# Autodesk Inventor assembly: Rack-RAM
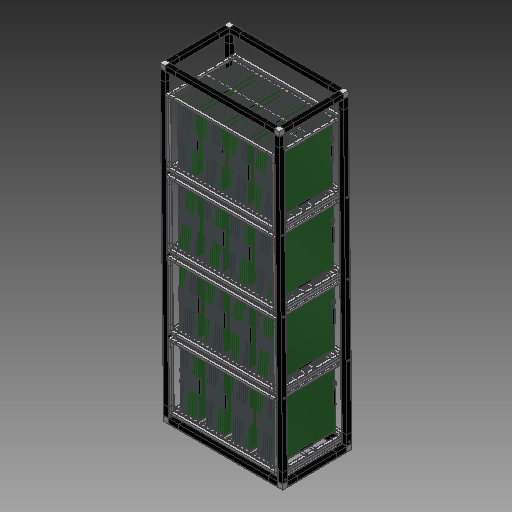
[picture p0: Inventor's stored thumbnail of the model, 512x512]
Saved by Autodesk Inventor 2018 (Build 220112000, 112)
## iProperties
Created: 2025-02-17
Part Number: Rack-RAM
Material: Všeobecné
Document SubType Name: Assembly
Designer: Jozko Mrkvicka
Author: Jozko Mrkvicka
## Documents named in this file (10)
- D:\05_Projekty\Projects_Inventor\Haluska9000\Rack-RAM.iam
- D:\05_Projekty\Projects_Inventor\Haluska9000\Profile-Connector\Profile-Connector#30x30xCorner.ipt
- D:\05_Projekty\Projects_Inventor\Haluska9000\Profile-Connector.ipt
- D:\05_Projekty\Projects_Inventor\Haluska9000\Cabinet-FerriteCore.iam
- D:\05_Projekty\Projects_Inventor\Haluska9000\Profile-Square-Black\Profile-Square#Rack-Ram-Height.ipt
- D:\05_Projekty\Projects_Inventor\Haluska9000\Profile-Square-Black.ipt
- D:\05_Projekty\Projects_Inventor\Haluska9000\Profile-Square-Black\Profile-Square#Rack-Ram-Width.ipt
- D:\05_Projekty\Projects_Inventor\Haluska9000\Profile-Square-Black\Profile-Square#Rack-Ram-Length.ipt
- D:\05_Projekty\Projects_Inventor\Haluska9000\Profile-T\Profile-T#Rack-Ram.ipt
- D:\05_Projekty\Projects_Inventor\Haluska9000\Profile-T.ipt
## Components (32 placed, 6 different names)
1. Cabinet-FerriteCore:1 [sub-assembly] — Proti sobě:627, Proti sobě:628, Stejný směr:50, Stejný směr:51
2. Profile-Connector#30x30xCorner:11 — Proti sobě:560, Proti sobě:561, Proti sobě:562, Proti sobě:572, Proti sobě:573, Proti sobě:574, Proti sobě:590, Proti sobě:591, Proti sobě:592
3. Profile-Connector#30x30xCorner:12 — Proti sobě:569, Proti sobě:570, Proti sobě:571, Proti sobě:575, Proti sobě:576, Proti sobě:577
4. Profile-Connector#30x30xCorner:13 — Proti sobě:581, Proti sobě:582, Proti sobě:583, Proti sobě:587, Proti sobě:588, Proti sobě:589
5. Profile-Connector#30x30xCorner:14 — Proti sobě:578, Proti sobě:579, Proti sobě:580, Proti sobě:584, Proti sobě:585, Proti sobě:586, Proti sobě:646, Proti sobě:647, Proti sobě:648
6. Profile-Square#Rack-Ram-Height:1 — Proti sobě:560, Proti sobě:561, Proti sobě:562, Proti sobě:581, Proti sobě:582, Proti sobě:583, Proti sobě:624, Stejný směr:36, Proti sobě:625, Stejný směr:40, Proti sobě:639, Proti sobě:640, Stejný směr:45, Stejný směr:46
7. Profile-Square#Rack-Ram-Height:3 — Proti sobě:569, Proti sobě:570, Proti sobě:571, Proti sobě:578, Proti sobě:579, Proti sobě:580, Proti sobě:623, Stejný směr:35, Proti sobě:626, Stejný směr:39, Proti sobě:629, Proti sobě:630, Proti sobě:637, Proti sobě:638, Stejný směr:43, Stejný směr:44, Proti sobě:641, Proti sobě:642
8. Profile-Square#Rack-Ram-Length:5 — Proti sobě:572, Proti sobě:573, Proti sobě:574, Proti sobě:620, Proti sobě:621, Proti sobě:622
9. Profile-Square#Rack-Ram-Length:6 — Proti sobě:575, Proti sobě:576, Proti sobě:577
10. Profile-Square#Rack-Ram-Length:11
11. Profile-Square#Rack-Ram-Length:12 — Proti sobě:646, Proti sobě:647, Proti sobě:648
12. Profile-Square#Rack-Ram-Width:7 — Proti sobě:584, Proti sobě:585, Proti sobě:586, Proti sobě:587, Proti sobě:588, Proti sobě:589
13. Profile-Square#Rack-Ram-Width:8 — Proti sobě:590, Proti sobě:591, Proti sobě:592
14. Profile-Square#Rack-Ram-Width:13
15. Profile-Square#Rack-Ram-Width:14 — Proti sobě:643, Proti sobě:644, Proti sobě:645
16. Profile-Connector#30x30xCorner:15
17. Profile-Connector#30x30xCorner:16 — Proti sobě:643, Proti sobě:644, Proti sobě:645
18. Profile-Connector#30x30xCorner:17 — Proti sobě:620, Proti sobě:621, Proti sobě:622, Proti sobě:631, Proti sobě:632, Proti sobě:633
19. Profile-Connector#30x30xCorner:18 — Proti sobě:634, Proti sobě:635, Proti sobě:636
20. Profile-T#Rack-Ram:1 — Proti sobě:623, Stejný směr:35, Stejný směr:37, Proti sobě:627, Proti sobě:628, Proti sobě:629
21. Profile-T#Rack-Ram:2 — Proti sobě:624, Stejný směr:36, Stejný směr:37
22. Profile-T#Rack-Ram:3 — Proti sobě:626, Stejný směr:39, Proti sobě:630, Proti sobě:649
23. Profile-T#Rack-Ram:4 — Proti sobě:625, Stejný směr:40
24. Profile-Square#Rack-Ram-Height:15 — Proti sobě:631, Proti sobě:632, Proti sobě:633
25. Profile-Square#Rack-Ram-Height:16 — Proti sobě:634, Proti sobě:635, Proti sobě:636
26. Profile-T#Rack-Ram:5 — Proti sobě:638, Stejný směr:43, Proti sobě:641, Proti sobě:650
27. Profile-T#Rack-Ram:6 — Proti sobě:640, Stejný směr:46
28. Profile-T#Rack-Ram:7 — Proti sobě:637, Stejný směr:44, Proti sobě:642, Proti sobě:651
29. Profile-T#Rack-Ram:8 — Proti sobě:639, Stejný směr:45
30. Cabinet-FerriteCore:2 [sub-assembly] — Proti sobě:650, Stejný směr:48, Stejný směr:49, Stejný směr:52, Stejný směr:53
31. Cabinet-FerriteCore:3 [sub-assembly] — Proti sobě:649, Stejný směr:49, Stejný směr:50, Stejný směr:51, Stejný směr:52
32. Cabinet-FerriteCore:4 [sub-assembly] — Proti sobě:651, Stejný směr:48, Stejný směr:53
## Relationships (92: Mate 74, Flush 18)
- Proti sobě:560 [Mate]: Profile-Connector#30x30xCorner:11 ↔ Profile-Square#Rack-Ram-Height:1
- Proti sobě:561 [Mate]: Profile-Connector#30x30xCorner:11 ↔ Profile-Square#Rack-Ram-Height:1
- Proti sobě:562 [Mate]: Profile-Connector#30x30xCorner:11 ↔ Profile-Square#Rack-Ram-Height:1
- Proti sobě:569 [Mate]: Profile-Connector#30x30xCorner:12 ↔ Profile-Square#Rack-Ram-Height:3
- Proti sobě:570 [Mate]: Profile-Connector#30x30xCorner:12 ↔ Profile-Square#Rack-Ram-Height:3
- Proti sobě:571 [Mate]: Profile-Connector#30x30xCorner:12 ↔ Profile-Square#Rack-Ram-Height:3
- Proti sobě:572 [Mate]: Profile-Connector#30x30xCorner:11 ↔ Profile-Square#Rack-Ram-Length:5
- Proti sobě:573 [Mate]: Profile-Connector#30x30xCorner:11 ↔ Profile-Square#Rack-Ram-Length:5
- Proti sobě:574 [Mate]: Profile-Connector#30x30xCorner:11 ↔ Profile-Square#Rack-Ram-Length:5
- Proti sobě:575 [Mate]: Profile-Connector#30x30xCorner:12 ↔ Profile-Square#Rack-Ram-Length:6
- Proti sobě:576 [Mate]: Profile-Connector#30x30xCorner:12 ↔ Profile-Square#Rack-Ram-Length:6
- Proti sobě:577 [Mate]: Profile-Connector#30x30xCorner:12 ↔ Profile-Square#Rack-Ram-Length:6
- Proti sobě:578 [Mate]: Profile-Connector#30x30xCorner:14 ↔ Profile-Square#Rack-Ram-Height:3
- Proti sobě:579 [Mate]: Profile-Connector#30x30xCorner:14 ↔ Profile-Square#Rack-Ram-Height:3
- Proti sobě:580 [Mate]: Profile-Connector#30x30xCorner:14 ↔ Profile-Square#Rack-Ram-Height:3
- Proti sobě:581 [Mate]: Profile-Connector#30x30xCorner:13 ↔ Profile-Square#Rack-Ram-Height:1
- Proti sobě:582 [Mate]: Profile-Connector#30x30xCorner:13 ↔ Profile-Square#Rack-Ram-Height:1
- Proti sobě:583 [Mate]: Profile-Connector#30x30xCorner:13 ↔ Profile-Square#Rack-Ram-Height:1
- Proti sobě:584 [Mate]: Profile-Connector#30x30xCorner:14 ↔ Profile-Square#Rack-Ram-Width:7
- Proti sobě:585 [Mate]: Profile-Connector#30x30xCorner:14 ↔ Profile-Square#Rack-Ram-Width:7
- Proti sobě:586 [Mate]: Profile-Connector#30x30xCorner:14 ↔ Profile-Square#Rack-Ram-Width:7
- Proti sobě:587 [Mate]: Profile-Connector#30x30xCorner:13 ↔ Profile-Square#Rack-Ram-Width:7
- Proti sobě:588 [Mate]: Profile-Connector#30x30xCorner:13 ↔ Profile-Square#Rack-Ram-Width:7
- Proti sobě:589 [Mate]: Profile-Connector#30x30xCorner:13 ↔ Profile-Square#Rack-Ram-Width:7
- Proti sobě:590 [Mate]: Profile-Connector#30x30xCorner:11 ↔ Profile-Square#Rack-Ram-Width:8
- Proti sobě:591 [Mate]: Profile-Connector#30x30xCorner:11 ↔ Profile-Square#Rack-Ram-Width:8
- Proti sobě:592 [Mate]: Profile-Connector#30x30xCorner:11 ↔ Profile-Square#Rack-Ram-Width:8
- [Mate]: Profile-Square#Rack-Ram-Length:11 ↔ Profile-Connector#30x30xCorner:15
- [Mate]: Profile-Square#Rack-Ram-Length:11 ↔ Profile-Connector#30x30xCorner:15
- [Mate]: Profile-Square#Rack-Ram-Length:11 ↔ Profile-Connector#30x30xCorner:15
- [Mate]: Profile-Square#Rack-Ram-Length:12 ↔ Profile-Connector#30x30xCorner:16
- [Mate]: Profile-Square#Rack-Ram-Length:12 ↔ Profile-Connector#30x30xCorner:16
- [Mate]: Profile-Square#Rack-Ram-Length:12 ↔ Profile-Connector#30x30xCorner:16
- [Mate]: Profile-Square#Rack-Ram-Width:13 ↔ Profile-Connector#30x30xCorner:18
- [Mate]: Profile-Square#Rack-Ram-Width:13 ↔ Profile-Connector#30x30xCorner:18
- [Mate]: Profile-Square#Rack-Ram-Width:13 ↔ Profile-Connector#30x30xCorner:18
- [Mate]: Profile-Square#Rack-Ram-Width:13 ↔ Profile-Connector#30x30xCorner:17
- [Mate]: Profile-Square#Rack-Ram-Width:13 ↔ Profile-Connector#30x30xCorner:17
- [Mate]: Profile-Square#Rack-Ram-Width:13 ↔ Profile-Connector#30x30xCorner:17
- [Mate]: Profile-Square#Rack-Ram-Width:14 ↔ Profile-Connector#30x30xCorner:15
- [Mate]: Profile-Square#Rack-Ram-Width:14 ↔ Profile-Connector#30x30xCorner:15
- [Mate]: Profile-Square#Rack-Ram-Width:14 ↔ Profile-Connector#30x30xCorner:15
- Proti sobě:620 [Mate]: Profile-Square#Rack-Ram-Length:5 ↔ Profile-Connector#30x30xCorner:17
- Proti sobě:621 [Mate]: Profile-Square#Rack-Ram-Length:5 ↔ Profile-Connector#30x30xCorner:17
- Proti sobě:622 [Mate]: Profile-Square#Rack-Ram-Length:5 ↔ Profile-Connector#30x30xCorner:17
- Proti sobě:623 [Mate]: Profile-Square#Rack-Ram-Height:3 ↔ Profile-T#Rack-Ram:1
- Stejný směr:35 [Flush]: Profile-Square#Rack-Ram-Height:3 ↔ Profile-T#Rack-Ram:1
- Proti sobě:624 [Mate]: Profile-Square#Rack-Ram-Height:1 ↔ Profile-T#Rack-Ram:2
- Stejný směr:36 [Flush]: Profile-Square#Rack-Ram-Height:1 ↔ Profile-T#Rack-Ram:2
- Stejný směr:37 [Flush]: Profile-T#Rack-Ram:1 ↔ Profile-T#Rack-Ram:2
- [Flush]: Profile-T#Rack-Ram:3 ↔ Profile-T#Rack-Ram:4
- Proti sobě:625 [Mate]: Profile-Square#Rack-Ram-Height:1 ↔ Profile-T#Rack-Ram:4
- Proti sobě:626 [Mate]: Profile-Square#Rack-Ram-Height:3 ↔ Profile-T#Rack-Ram:3
- Stejný směr:39 [Flush]: Profile-Square#Rack-Ram-Height:3 ↔ Profile-T#Rack-Ram:3
- Stejný směr:40 [Flush]: Profile-Square#Rack-Ram-Height:1 ↔ Profile-T#Rack-Ram:4
- Proti sobě:627 [Mate]: Cabinet-FerriteCore:1 ↔ Profile-T#Rack-Ram:1
- Proti sobě:628 [Mate] (1 mm): Cabinet-FerriteCore:1 ↔ Profile-T#Rack-Ram:1
- Proti sobě:629 [Mate]: Profile-Square#Rack-Ram-Height:3 ↔ Profile-T#Rack-Ram:1
- Proti sobě:630 [Mate]: Profile-Square#Rack-Ram-Height:3 ↔ Profile-T#Rack-Ram:3
- Proti sobě:631 [Mate]: Profile-Connector#30x30xCorner:17 ↔ Profile-Square#Rack-Ram-Height:15
- Proti sobě:632 [Mate]: Profile-Connector#30x30xCorner:17 ↔ Profile-Square#Rack-Ram-Height:15
- Proti sobě:633 [Mate]: Profile-Connector#30x30xCorner:17 ↔ Profile-Square#Rack-Ram-Height:15
- Proti sobě:634 [Mate]: Profile-Connector#30x30xCorner:18 ↔ Profile-Square#Rack-Ram-Height:16
- Proti sobě:635 [Mate]: Profile-Connector#30x30xCorner:18 ↔ Profile-Square#Rack-Ram-Height:16
- Proti sobě:636 [Mate]: Profile-Connector#30x30xCorner:18 ↔ Profile-Square#Rack-Ram-Height:16
- [Flush]: Profile-T#Rack-Ram:5 ↔ Profile-T#Rack-Ram:6
- [Flush]: Profile-T#Rack-Ram:7 ↔ Profile-T#Rack-Ram:8
- Proti sobě:637 [Mate]: Profile-Square#Rack-Ram-Height:3 ↔ Profile-T#Rack-Ram:7
- Proti sobě:638 [Mate]: Profile-Square#Rack-Ram-Height:3 ↔ Profile-T#Rack-Ram:5
- Proti sobě:639 [Mate]: Profile-Square#Rack-Ram-Height:1 ↔ Profile-T#Rack-Ram:8
- Proti sobě:640 [Mate]: Profile-Square#Rack-Ram-Height:1 ↔ Profile-T#Rack-Ram:6
- Stejný směr:43 [Flush]: Profile-Square#Rack-Ram-Height:3 ↔ Profile-T#Rack-Ram:5
- Stejný směr:44 [Flush]: Profile-Square#Rack-Ram-Height:3 ↔ Profile-T#Rack-Ram:7
- Stejný směr:45 [Flush]: Profile-Square#Rack-Ram-Height:1 ↔ Profile-T#Rack-Ram:8
- Stejný směr:46 [Flush]: Profile-Square#Rack-Ram-Height:1 ↔ Profile-T#Rack-Ram:6
- Proti sobě:641 [Mate]: Profile-Square#Rack-Ram-Height:3 ↔ Profile-T#Rack-Ram:5
- Proti sobě:642 [Mate]: Profile-Square#Rack-Ram-Height:3 ↔ Profile-T#Rack-Ram:7
- Proti sobě:643 [Mate]: Profile-Square#Rack-Ram-Width:14 ↔ Profile-Connector#30x30xCorner:16
- Proti sobě:644 [Mate]: Profile-Square#Rack-Ram-Width:14 ↔ Profile-Connector#30x30xCorner:16
- Proti sobě:645 [Mate]: Profile-Square#Rack-Ram-Width:14 ↔ Profile-Connector#30x30xCorner:16
- Proti sobě:646 [Mate]: Profile-Connector#30x30xCorner:14 ↔ Profile-Square#Rack-Ram-Length:12
- Proti sobě:647 [Mate]: Profile-Connector#30x30xCorner:14 ↔ Profile-Square#Rack-Ram-Length:12
- Proti sobě:648 [Mate]: Profile-Connector#30x30xCorner:14 ↔ Profile-Square#Rack-Ram-Length:12
- Proti sobě:649 [Mate]: Profile-T#Rack-Ram:3 ↔ Cabinet-FerriteCore:3
- Proti sobě:650 [Mate]: Profile-T#Rack-Ram:5 ↔ Cabinet-FerriteCore:2
- Proti sobě:651 [Mate]: Profile-T#Rack-Ram:7 ↔ Cabinet-FerriteCore:4
- Stejný směr:48 [Flush]: Cabinet-FerriteCore:2 ↔ Cabinet-FerriteCore:4
- Stejný směr:49 [Flush]: Cabinet-FerriteCore:2 ↔ Cabinet-FerriteCore:3
- Stejný směr:50 [Flush]: Cabinet-FerriteCore:1 ↔ Cabinet-FerriteCore:3
- Stejný směr:51 [Flush]: Cabinet-FerriteCore:1 ↔ Cabinet-FerriteCore:3
- Stejný směr:52 [Flush]: Cabinet-FerriteCore:2 ↔ Cabinet-FerriteCore:3
- Stejný směr:53 [Flush]: Cabinet-FerriteCore:2 ↔ Cabinet-FerriteCore:4
## Named parameters: d1044_d1033 = 0 mm, d1045_d1034 = 0 mm, d1046_d1035 = 0 mm, d1047_d1036 = 0 mm, d1048_d1037 = 0 mm, d1049_d1038 = 0 mm, d1050_d1039 = 0 mm, d1051_d1040 = 0 mm, d1052_d1041 = 0 mm, d1059_d1021 = 0 mm, d1060_d1022 = 0 mm, d1061_d1023 = 0 mm, d1062_d1024 = 0 mm, d1063_d1025 = 0 mm, d1064_d1026 = 0 mm, d1077_d1076 = 0 mm, d1092_d1077_d1076 = 0 mm, d1093_d1077_d1076 = 0 mm
